# Autodesk Inventor assembly: UBG-Rad Getriebe
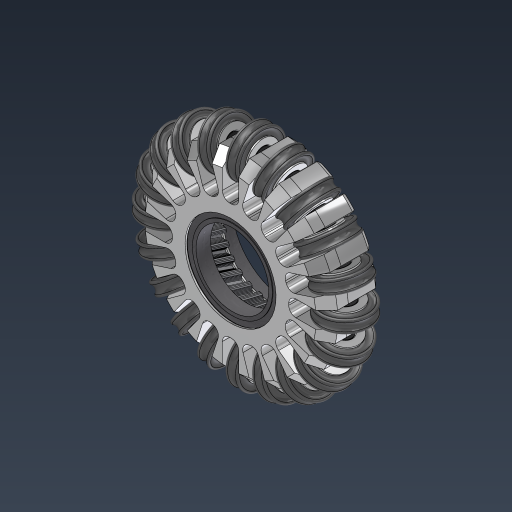
[picture p0: Inventor's stored thumbnail of the model, 512x512]
Saved by Autodesk Inventor 2023.1 (Build 271208000, 208)
## iProperties
Part Number: UBG-Rad Getriebe
Material: Generisch
Document SubType Name: Assembly
Designer: rYan
Mass: 53.555 g
Surface Area: 435.52 cm^2
Volume: 34.2485 cm^3
Density: 1.56372 g/cm^3
Author: rYan
## Documents named in this file (7)
- D:\TIGERsGIT\Hardware\mechanik\2024\Inventor\Robot\Drive Train\Geared\UBG-Rad Getriebe.iam
- D:\TIGERsGIT\Hardware\mechanik\2024\Inventor\Robot\Drive Train\Geared\Radkasten Getriebe.ipt
- D:\TIGERsGIT\Hardware\mechanik\2024\Inventor\Robot\Drive Train\Common\MG-Rolle.iam
- D:\TIGERsGIT\Hardware\mechanik\2024\Inventor\Robot\Drive Train\Geared\Raddeckel Getriebe.ipt
- D:\TIGERsGIT\Hardware\mechanik\2024\Inventor\Robot\Drive Train\Geared\Planetengetriebe Hohlrad.ipt
- D:\TIGERsGIT\Hardware\mechanik\2024\Inventor\Purchased Parts\Kugellager 6704-ZZ.ipt
- D:\TIGERsGIT\Hardware\mechanik\2024\Inventor\Purchased Parts\Kugellager 6706-2RS.ipt
## Components (25 placed, 6 different names)
1. Radkasten:1 — Fluchtend:1, Fluchtend:2, Passend:5, Passend:11, Passend:14, Fluchtend:4, Fluchtend:5, Fluchtend:6, Einfügen:20, Einfügen:22, Passend:15
2. Raddeckel:1 — Passend:10, Passend:14, Einfügen:16, Fluchtend:5, Fluchtend:6
3. Kugellager 6704-ZZ:1 — Einfügen:16
4. Planetengetriebe Hohlrad z23:1 — Einfügen:22, Passend:15
5. Kugellager 6706-2RS:1 — Einfügen:20
6. MG-Rolle:1 [sub-assembly] — Passend:2, Winkel:1, Passend:6, Passend:12
7. MG-Rolle:2 [sub-assembly]
8. MG-Rolle:3 [sub-assembly]
9. MG-Rolle:4 [sub-assembly]
10. MG-Rolle:5 [sub-assembly]
11. MG-Rolle:6 [sub-assembly]
12. MG-Rolle:7 [sub-assembly]
13. MG-Rolle:8 [sub-assembly]
14. MG-Rolle:9 [sub-assembly]
15. MG-Rolle:10 [sub-assembly]
16. MG-Rolle:11 [sub-assembly]
17. MG-Rolle:12 [sub-assembly]
18. MG-Rolle:13 [sub-assembly]
19. MG-Rolle:14 [sub-assembly]
20. MG-Rolle:15 [sub-assembly]
21. MG-Rolle:16 [sub-assembly]
22. MG-Rolle:17 [sub-assembly]
23. MG-Rolle:18 [sub-assembly]
24. MG-Rolle:19 [sub-assembly]
25. MG-Rolle:20 [sub-assembly]
## Component patterns: (20 elements, first: MG-Rolle:1)
## Relationships (19: Mate 8, Flush 6, Insert 3, Angle 2)
- Fluchtend:1 [Flush]: Radkasten:1
- Fluchtend:2 [Flush]: Radkasten:1
- Passend:2 [Mate]: MG-Rolle:1
- Winkel:1 [Angle] (0 deg): MG-Rolle:1
- Passend:5 [Mate]: Radkasten:1
- Passend:6 [Mate]: MG-Rolle:1
- Fluchtend:3 [Flush] (31.3 mm)
- Passend:10 [Mate]: Raddeckel:1
- Winkel:2 [Angle] (0 deg)
- Passend:11 [Mate]: Radkasten:1
- Passend:12 [Mate]: MG-Rolle:1
- Passend:14 [Mate]: Radkasten:1 ↔ Raddeckel:1
- Einfügen:16 [Insert]: Raddeckel:1 ↔ Kugellager 6704-ZZ:1
- Fluchtend:4 [Flush]: Radkasten:1
- Fluchtend:5 [Flush]: Radkasten:1 ↔ Raddeckel:1
- Fluchtend:6 [Flush]: Radkasten:1 ↔ Raddeckel:1
- Einfügen:20 [Insert]: Radkasten:1 ↔ Kugellager 6706-2RS:1
- Einfügen:22 [Insert]: Radkasten:1 ↔ Planetengetriebe Hohlrad z23:1
- Passend:15 [Mate]: Radkasten:1 ↔ Planetengetriebe Hohlrad z23:1
